# Autodesk Inventor assembly: 한쪽발받침대
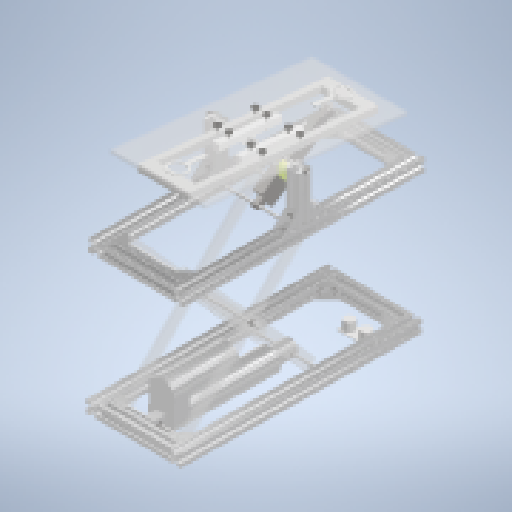
[picture p0: Inventor's stored thumbnail of the model, 512x512]
Saved by Autodesk Inventor 2024 (Build 280153000, 153)
## iProperties
Created: 2024-04-15
Part Number: 한쪽발받침대
Document SubType Name: Assembly
Designer: kkamin5
Mass: 2729.98 g
Surface Area: 7750.02 cm^2
Volume: 1186.1 cm^3
Density: 2.30165 g/cm^3
Author: kkamin5
## Documents named in this file (31)
- C:\Users\kkamin5\OneDrive - UOS\문서\Inventor\EBS project\모델링최종\한쪽발받침대.iam
- C:\Users\kkamin5\OneDrive - UOS\문서\Inventor\EBS project\모델링최종\프로파일_110.ipt
- C:\Users\kkamin5\OneDrive - UOS\문서\Inventor\EBS project\모델링최종\프로파일_380.ipt
- C:\Users\kkamin5\OneDrive - UOS\문서\Inventor\EBS project\모델링최종\t형 슬라이더.ipt
- C:\Users\kkamin5\OneDrive - UOS\문서\Inventor\EBS project\모델링최종\L형 브라켓.ipt
- C:\Users\kkamin5\OneDrive - UOS\문서\Inventor\EBS project\모델링최종\x바.ipt
- C:\Users\kkamin5\OneDrive - UOS\문서\Inventor\EBS project\모델링최종\프로파일_80.ipt
- C:\Users\kkamin5\OneDrive - UOS\문서\Inventor\EBS project\모델링최종\회전체_3d프린트.ipt
- C:\Users\kkamin5\OneDrive - UOS\문서\Inventor\EBS project\모델링최종\발판.ipt
- C:\Users\kkamin5\OneDrive - UOS\문서\Inventor\EBS project\모델링최종\각도엑추에이터브라켓.ipt
- C:\Users\kkamin5\OneDrive - UOS\문서\Inventor\EBS project\모델링최종\120mm 4M 볼트.ipt
- C:\Users\kkamin5\OneDrive - UOS\문서\Inventor\EBS project\모델링최종\볼트M4 10mm.ipt
- C:\Users\kkamin5\OneDrive - UOS\문서\Inventor\EBS project\모델링최종\L브래킷_T슬라이드 볼트조임.iam
- C:\Users\kkamin5\OneDrive - UOS\문서\Inventor\Content Center Files\R2024\ko-KR\BS EN 24035\ISO 4035 - M4BS EN.ipt
- C:\Users\kkamin5\OneDrive - UOS\문서\Inventor\EBS project\모델링최종\M4 볼트 150mm.ipt
- C:\Users\kkamin5\OneDrive - UOS\문서\Inventor\Content Center Files\R2024\ko-KR\ANSI B 18.2.4.1 M(1)\ANSI B 18.2.4.1 M - M4 x 0.7Style 1.ipt
- C:\Users\kkamin5\OneDrive - UOS\문서\Inventor\EBS project\모델링최종\M4 볼트 15mm.ipt
- C:\Users\kkamin5\OneDrive - UOS\문서\Inventor\EBS project\모델링최종\초음파센서.ipt
- C:\Users\kkamin5\OneDrive - UOS\문서\Inventor\EBS project\모델링최종\평기어_가변저항.ipt
- C:\Users\kkamin5\OneDrive - UOS\문서\Inventor\EBS project\모델링최종\각도조절 액추에이터_중간.ipt
- C:\Users\kkamin5\OneDrive - UOS\문서\Inventor\EBS project\모델링최종\높이조절 액추에이터_최소.ipt
- C:\Users\kkamin5\OneDrive - UOS\문서\Inventor\EBS project\모델링최종\압력센서.ipt
- C:\Users\kkamin5\OneDrive - UOS\문서\Inventor\EBS project\모델링최종\가변저항.ipt
- C:\Users\kkamin5\OneDrive - UOS\문서\Inventor\EBS project\모델링최종\초음파센서거리측정용아크릴판.ipt
- C:\Users\kkamin5\OneDrive - UOS\문서\Inventor\EBS project\모델링최종\발판보강지지대2.ipt
- C:\Users\kkamin5\OneDrive - UOS\문서\Inventor\EBS project\모델링최종\한쪽발받침대\AIP\FEA\eo59sf0n4.fins
- C:\Users\kkamin5\OneDrive - UOS\문서\Inventor\EBS project\모델링최종\한쪽발받침대\AIP\FEA\eo59sf0n4.fsat
- C:\Users\kkamin5\OneDrive - UOS\문서\Inventor\EBS project\모델링최종\한쪽발받침대\AIP\FEA\eo59sf0n4.ftes
- C:\Users\kkamin5\OneDrive - UOS\문서\Inventor\EBS project\모델링최종\한쪽발받침대\AIP\FEA\eo59sf0n4.fwiz
- C:\Users\kkamin5\OneDrive - UOS\문서\Inventor\EBS project\모델링최종\한쪽발받침대\AIP\FEA\eo59sf0tc.fmsh
- C:\Users\kkamin5\OneDrive - UOS\문서\Inventor\EBS project\모델링최종\한쪽발받침대\AIP\FEA\eo5b5hja8.fres
## Components (100 placed, 24 different names)
1. 프로파일_110:1 — 메이트:132, 메이트:133, 메이트:134, 메이트:135, 메이트:144
2. 프로파일_380:1 — 메이트:136, 메이트:138, 메이트:148, 플러쉬:34, 플러쉬:52, 메이트:327, 메이트:328
3. 프로파일_110:2 — 메이트:146, 플러쉬:33, 메이트:149, 메이트:265
4. 프로파일_380:2 — 메이트:137, 메이트:147
5. 프로파일_110:3
6. 프로파일_380:3 — 메이트:161, 메이트:162, 메이트:164, 메이트:166, 메이트:190, 메이트:335
7. 프로파일_110:4 — 메이트:189, 플러쉬:40, 메이트:191, 플러쉬:41, 메이트:341
8. 프로파일_380:4 — 메이트:169, 메이트:170, 플러쉬:39, 메이트:176, 메이트:192, 메이트:340
9. t형 슬라이더:1 — 메이트:139
10. t형 슬라이더:2 — 메이트:174
11. t형 슬라이더:3 — 메이트:198
12. t형 슬라이더:4 — 메이트:175
13. t형 슬라이더:5 — 메이트:129
14. t형 슬라이더:6 — 메이트:131
15. x바:1 — 메이트:130, 메이트:160, 메이트:182
16. x바:2 — 메이트:126, 메이트:141, 메이트:159, 메이트:185
17. x바:3 — 메이트:125, 메이트:140, 메이트:188
18. x바:4 — 메이트:128, 메이트:142, 메이트:179
19. t형 슬라이더:7
20. t형 슬라이더:8 — 메이트:163
21. t형 슬라이더:9 — 메이트:173, 플러쉬:42
22. t형 슬라이더:10 — 메이트:172
23. 프로파일_80:1 — 메이트:168, 플러쉬:38, 메이트:171, 플러쉬:42, 플러쉬:47, 메이트:219
24. 프로파일_80:2 — 플러쉬:36, 메이트:165, 메이트:167, 플러쉬:37, 메이트:215, 메이트:217, 메이트:330, 메이트:333, 각도:3, 플러쉬:56
25. L형 브라켓:5 — 메이트:152, 메이트:153, 메이트:154
26. L형 브라켓:6 — 메이트:143, 메이트:156, 메이트:157
27. L형 브라켓:7 — 메이트:237, 메이트:238, 메이트:239
28. L형 브라켓:8 — 메이트:234, 메이트:235, 메이트:236
29. 회전체_3d프린트:1 — 메이트:209, 메이트:311, 메이트:312, 메이트:317, 메이트:318, 메이트:338
30. 발판:1 — 메이트:214, 플러쉬:48, 플러쉬:49, 메이트:269, 메이트:278, 메이트:281, 플러쉬:56, 메이트:344
31. 각도엑추에이터브라켓:1 — 메이트:229, 메이트:245, 메이트:259, 메이트:323
32. 120mm 4M 볼트:1 — 메이트:125, 메이트:126, 메이트:138, 메이트:139, 메이트:184, 메이트:187, 메이트:198, 메이트:256, 메이트:257, 메이트:320
33. 120mm 4M 볼트:2 — 메이트:128, 메이트:129, 메이트:130, 메이트:131, 메이트:136, 메이트:137, 메이트:143, 메이트:178, 메이트:181, 메이트:210, 메이트:211, 메이트:319
34. t형 슬라이더:11 — 메이트:132, 메이트:133, 메이트:158
35. t형 슬라이더:12 — 메이트:134, 메이트:135, 메이트:145
36. 120mm 4M 볼트:3 — 메이트:140, 메이트:141, 메이트:142, 메이트:250, 메이트:251, 메이트:324
37. 볼트M4 10mm:1 — 메이트:144, 메이트:145, 메이트:155, 메이트:157, 메이트:158
38. L브래킷_T슬라이드 볼트조임:1 [sub-assembly] — 메이트:146, 메이트:147, 플러쉬:33
39. L브래킷_T슬라이드 볼트조임:2 [sub-assembly] — 메이트:148, 메이트:149, 플러쉬:34
40. t형 슬라이더:13 — 메이트:152
41. 볼트M4 10mm:2 — 메이트:154
42. BS EN 24035 - 미터 M4:1 — 메이트:153
43. BS EN 24035 - 미터 M4:2 — 메이트:155, 메이트:156
44. 120mm 4M 볼트:4 — 메이트:159, 메이트:162, 메이트:163, 메이트:183, 메이트:186
45. 120mm 4M 볼트:5 — 메이트:160, 메이트:161, 메이트:174, 메이트:175, 메이트:177, 메이트:180
46. L브래킷_T슬라이드 볼트조임:3 [sub-assembly] — 메이트:189, 메이트:190, 플러쉬:40, 메이트:339
47. L브래킷_T슬라이드 볼트조임:4 [sub-assembly] — 메이트:170, 메이트:171, 플러쉬:39
48. L브래킷_T슬라이드 볼트조임:5 [sub-assembly] — 메이트:168, 메이트:169, 플러쉬:38
49. L브래킷_T슬라이드 볼트조임:6 [sub-assembly] — 메이트:166, 메이트:167, 플러쉬:37
50. L브래킷_T슬라이드 볼트조임:7 [sub-assembly] — 메이트:191, 메이트:192, 플러쉬:41
51. L브래킷_T슬라이드 볼트조임:8 [sub-assembly] — 플러쉬:36, 메이트:164, 메이트:165
52. 120mm 4M 볼트:6 — 메이트:172, 메이트:173, 메이트:176, 메이트:321
53. x바:5 — 메이트:177, 메이트:178, 메이트:179, 메이트:252, 메이트:324
54. x바:6 — 메이트:180, 메이트:181, 메이트:182, 메이트:253
55. x바:7 — 메이트:183, 메이트:184, 메이트:185
56. x바:8 — 메이트:186, 메이트:187, 메이트:188
57. M4 볼트 150mm:1 — 메이트:209, 플러쉬:47, 메이트:215, 메이트:216, 메이트:218, 메이트:272
58. 6각 너트 미터 M4 x 0.7:1 — 메이트:211, 메이트:326
59. 6각 너트 미터 M4 x 0.7:2 — 메이트:210, 메이트:325, 메이트:327
60. 발판:2 — 메이트:214, 플러쉬:48, 플러쉬:49, 메이트:284, 메이트:285, 메이트:288, 메이트:289, 메이트:292, 메이트:293, 메이트:296, 메이트:297, 메이트:303, 메이트:304, 메이트:305, 메이트:306, 메이트:307, 메이트:308, 메이트:309, 메이트:310, 메이트:331, 메이트:332, 각도:1, 각도:2
61. 6각 너트 미터 M4 x 0.7:3 — 메이트:218, 메이트:219
62. 6각 너트 미터 M4 x 0.7:4 — 메이트:216, 메이트:217
63. M4 볼트 15mm:5 — 메이트:229, 메이트:244, 메이트:259, 메이트:322
64. t형 슬라이더:14 — 메이트:235
65. 볼트M4 10mm:3 — 메이트:236
66. BS EN 24035 - 미터 M4:3 — 메이트:234
67. t형 슬라이더:15 — 메이트:237
68. 볼트M4 10mm:4 — 메이트:239
69. BS EN 24035 - 미터 M4:4 — 메이트:238
70. BS EN 24035 - 미터 M4:5 — 메이트:244, 메이트:245
71. BS EN 24035 - 미터 M4:10 — 메이트:250, 메이트:253
72. BS EN 24035 - 미터 M4:11 — 메이트:251, 메이트:252
73. BS EN 24035 - 미터 M4:14 — 메이트:256, 메이트:329
74. BS EN 24035 - 미터 M4:15 — 메이트:257, 메이트:328, 메이트:329
75. 초음파센서:2 — 플러쉬:52, 메이트:265
76. 회전체_3d프린트:2 — 메이트:269, 메이트:272, 메이트:278, 메이트:281, 메이트:286, 메이트:290, 메이트:336, 메이트:337
77. M4 볼트 15mm:6 — 메이트:284, 메이트:285
78. BS EN 24035 - 미터 M4:16 — 메이트:286
79. M4 볼트 15mm:7 — 메이트:288, 메이트:289
80. BS EN 24035 - 미터 M4:17 — 메이트:290
81. M4 볼트 15mm:8 — 메이트:292, 메이트:293
82. BS EN 24035 - 미터 M4:18
83. M4 볼트 15mm:9 — 메이트:296, 메이트:297
84. BS EN 24035 - 미터 M4:19
85. M4 볼트 15mm:10 — 메이트:299, 메이트:303, 메이트:307, 메이트:318
86. BS EN 24035 - 미터 M4:20 — 메이트:299, 메이트:311
87. M4 볼트 15mm:11 — 메이트:304, 메이트:308, 메이트:342
88. BS EN 24035 - 미터 M4:21
89. M4 볼트 15mm:12 — 메이트:305, 메이트:309, 메이트:317
90. BS EN 24035 - 미터 M4:22 — 메이트:312
91. M4 볼트 15mm:13 — 메이트:306, 메이트:310, 메이트:343
92. BS EN 24035 - 미터 M4:23
93. 평기어_가변저항:1 — 메이트:330, 메이트:334
94. 각도조절 액추에이터_중간:1 — 메이트:321, 메이트:322, 메이트:323
95. 높이조절 액추에이터_최소:1 — 메이트:319, 메이트:320, 메이트:325, 메이트:326
96. 압력센서:1 — 메이트:332, 각도:2, 플러쉬:55, 메이트:338
97. 압력센서:2 — 메이트:331, 각도:1, 플러쉬:55, 메이트:336, 메이트:337
98. 가변저항:1 — 메이트:333, 메이트:334, 각도:3, 메이트:335
99. 초음파센서거리측정용아크릴판:1 — 메이트:339, 메이트:340, 메이트:341
100. 발판보강지지대2:1 — 메이트:342, 메이트:343, 메이트:344
## Relationships (246: Mate 202, Flush 41, Angle 3)
- [Mate]: 프로파일_110:2 ↔ 프로파일_380:2
- [Flush]: 프로파일_110:2 ↔ 프로파일_380:2
- [Flush]: 프로파일_110:2 ↔ 프로파일_380:2
- [Mate]: 프로파일_380:1 ↔ 프로파일_110:2
- [Flush]: 프로파일_380:1 ↔ 프로파일_110:2
- [Flush]: 프로파일_380:1 ↔ 프로파일_110:2
- [Mate]: 프로파일_110:1 ↔ 프로파일_380:1
- [Flush]: 프로파일_110:1 ↔ 프로파일_380:1
- [Flush]: 프로파일_110:1 ↔ 프로파일_380:1
- [Mate]: 프로파일_110:4 ↔ 프로파일_380:4
- [Flush]: 프로파일_110:4 ↔ 프로파일_380:4
- [Flush]: 프로파일_110:4 ↔ 프로파일_380:4
- [Mate]: 프로파일_380:3 ↔ 프로파일_110:4
- [Flush]: 프로파일_380:3 ↔ 프로파일_110:4
- [Flush]: 프로파일_380:3 ↔ 프로파일_110:4
- [Mate]: 프로파일_110:3 ↔ 프로파일_380:3
- [Flush]: 프로파일_110:3 ↔ 프로파일_380:3
- [Flush]: 프로파일_110:3 ↔ 프로파일_380:3
- [Mate] (0.4 mm): 프로파일_380:4 ↔ t형 슬라이더:4
- [Mate] (0.1 mm): 프로파일_380:4 ↔ t형 슬라이더:4
- [Mate] (0.4 mm): 프로파일_380:2 ↔ t형 슬라이더:3
- [Mate] (0.2 mm): 프로파일_380:2 ↔ t형 슬라이더:3
- [Mate] (0.4 mm): 프로파일_380:3 ↔ t형 슬라이더:2
- [Mate] (0.1 mm): 프로파일_380:3 ↔ t형 슬라이더:2
- [Mate] (0.4 mm): 프로파일_380:1 ↔ t형 슬라이더:1
- [Mate]: 프로파일_380:1 ↔ t형 슬라이더:1
- [Flush]: 프로파일_110:1 ↔ 프로파일_110:3
- [Flush]: 프로파일_380:1 ↔ 프로파일_380:3
- [Mate] (0.4 mm): 프로파일_380:2 ↔ t형 슬라이더:6
- [Mate] (0.1 mm): 프로파일_380:2 ↔ t형 슬라이더:6
- [Mate] (0.4 mm): 프로파일_380:1 ↔ t형 슬라이더:5
- [Mate] (0.1 mm): 프로파일_380:1 ↔ t형 슬라이더:5
- [Mate]: x바:1 ↔ x바:4
- [Mate] (10 mm): 프로파일_380:4 ↔ x바:1
- [Mate] (10 mm): 프로파일_380:3 ↔ x바:4
- [Mate] (0.4 mm): 프로파일_380:4 ↔ t형 슬라이더:7
- [Mate]: 프로파일_380:4 ↔ t형 슬라이더:7
- [Mate]: 프로파일_380:3 ↔ t형 슬라이더:8
- [Mate]: 프로파일_380:3 ↔ t형 슬라이더:8
- [Flush]: t형 슬라이더:6 ↔ t형 슬라이더:7
- [Mate] (14 mm): 프로파일_380:1 ↔ x바:3
- [Mate] (14 mm): 프로파일_380:2 ↔ x바:2
- [Mate]: 프로파일_380:4 ↔ t형 슬라이더:9
- [Mate] (0.4 mm): 프로파일_380:4 ↔ t형 슬라이더:9
- [Mate]: 프로파일_380:3 ↔ t형 슬라이더:10
- [Mate] (0.4 mm): 프로파일_380:3 ↔ t형 슬라이더:10
- [Mate]: 프로파일_380:3 ↔ 프로파일_80:2
- [Mate]: 프로파일_380:4 ↔ 프로파일_80:1
- [Flush]: 프로파일_380:4 ↔ 프로파일_80:1
- [Flush]: 프로파일_380:3 ↔ 프로파일_80:2
- [Flush] (180 mm): 프로파일_380:4 ↔ 프로파일_80:1
- [Flush] (5 mm): t형 슬라이더:10 ↔ 프로파일_80:2
- [Mate]: 프로파일_380:2 ↔ L형 브라켓:5
- [Flush] (1.5 mm): 프로파일_110:1 ↔ L형 브라켓:5
- [Mate]: 프로파일_110:1 ↔ L형 브라켓:5
- [Mate]: 프로파일_380:1 ↔ L형 브라켓:6
- [Flush] (1.5 mm): 프로파일_110:1 ↔ L형 브라켓:6
- [Mate]: 프로파일_110:1 ↔ L형 브라켓:6
- [Flush] (1.5 mm): 프로파일_110:3 ↔ L형 브라켓:7
- [Mate]: 프로파일_380:3 ↔ L형 브라켓:7
- [Mate]: 프로파일_110:3 ↔ L형 브라켓:7
- [Flush] (1.5 mm): 프로파일_110:3 ↔ L형 브라켓:8
- [Mate]: 프로파일_110:3 ↔ L형 브라켓:8
- [Mate]: 프로파일_380:4 ↔ L형 브라켓:8
- [Mate]: 회전체_3d프린트:1 ↔ 발판:1
- [Mate]: 발판:1 ↔ 각도엑추에이터브라켓:1
- [Mate]: 발판:1 ↔ 각도엑추에이터브라켓:1
- 메이트:125 [Mate]: x바:3 ↔ 120mm 4M 볼트:1
- 메이트:126 [Mate]: x바:2 ↔ 120mm 4M 볼트:1
- 메이트:128 [Mate]: x바:4 ↔ 120mm 4M 볼트:2
- 메이트:129 [Mate]: t형 슬라이더:5 ↔ 120mm 4M 볼트:2
- 메이트:130 [Mate]: x바:1 ↔ 120mm 4M 볼트:2
- 메이트:131 [Mate]: t형 슬라이더:6 ↔ 120mm 4M 볼트:2
- 메이트:132 [Mate] (0.1 mm): 프로파일_110:1 ↔ t형 슬라이더:11
- 메이트:133 [Mate] (0.4 mm): 프로파일_110:1 ↔ t형 슬라이더:11
- 메이트:134 [Mate] (0.4 mm): 프로파일_110:1 ↔ t형 슬라이더:12
- 메이트:135 [Mate] (0.1 mm): 프로파일_110:1 ↔ t형 슬라이더:12
- 메이트:136 [Mate] (1 mm): 프로파일_380:1 ↔ 120mm 4M 볼트:2
- 메이트:137 [Mate] (1 mm): 프로파일_380:2 ↔ 120mm 4M 볼트:2
- 메이트:138 [Mate] (1 mm): 프로파일_380:1 ↔ 120mm 4M 볼트:1
- 메이트:139 [Mate]: t형 슬라이더:1 ↔ 120mm 4M 볼트:1
- 메이트:140 [Mate]: x바:3 ↔ 120mm 4M 볼트:3
- 메이트:141 [Mate]: x바:2 ↔ 120mm 4M 볼트:3
- 메이트:142 [Mate]: x바:4 ↔ 120mm 4M 볼트:3
- 메이트:143 [Mate]: L형 브라켓:6 ↔ 120mm 4M 볼트:2
- 메이트:144 [Mate]: 프로파일_110:1 ↔ 볼트M4 10mm:1
- 메이트:145 [Mate]: t형 슬라이더:12 ↔ 볼트M4 10mm:1
- 메이트:146 [Mate]: 프로파일_110:2 ↔ L브래킷_T슬라이드 볼트조임:1
- 메이트:147 [Mate]: 프로파일_380:2 ↔ L브래킷_T슬라이드 볼트조임:1
- 플러쉬:33 [Flush] (1.5 mm): 프로파일_110:2 ↔ L브래킷_T슬라이드 볼트조임:1
- 메이트:148 [Mate]: 프로파일_380:1 ↔ L브래킷_T슬라이드 볼트조임:2
- 메이트:149 [Mate]: 프로파일_110:2 ↔ L브래킷_T슬라이드 볼트조임:2
- 플러쉬:34 [Flush] (1.5 mm): 프로파일_380:1 ↔ L브래킷_T슬라이드 볼트조임:2
- [Mate]: t형 슬라이더:13 ↔ 볼트M4 10mm:2
- [Flush]: t형 슬라이더:13 ↔ 볼트M4 10mm:2
- [Mate]: 볼트M4 10mm:2 ↔ BS EN 24035 - 미터 M4:1
- 메이트:152 [Mate] (1.6 mm): L형 브라켓:5 ↔ t형 슬라이더:13
- 메이트:153 [Mate]: L형 브라켓:5 ↔ BS EN 24035 - 미터 M4:1
- 메이트:154 [Mate]: L형 브라켓:5 ↔ 볼트M4 10mm:2
- 메이트:155 [Mate]: 볼트M4 10mm:1 ↔ BS EN 24035 - 미터 M4:2
- 메이트:156 [Mate]: L형 브라켓:6 ↔ BS EN 24035 - 미터 M4:2
- 메이트:157 [Mate]: L형 브라켓:6 ↔ 볼트M4 10mm:1
- 메이트:158 [Mate]: t형 슬라이더:11 ↔ 볼트M4 10mm:1
- 메이트:159 [Mate]: x바:2 ↔ 120mm 4M 볼트:4
- 메이트:160 [Mate]: x바:1 ↔ 120mm 4M 볼트:5
- 메이트:161 [Mate] (1 mm): 프로파일_380:3 ↔ 120mm 4M 볼트:5
- 메이트:162 [Mate] (1 mm): 프로파일_380:3 ↔ 120mm 4M 볼트:4
- 메이트:163 [Mate]: t형 슬라이더:8 ↔ 120mm 4M 볼트:4
- 플러쉬:36 [Flush] (1.5 mm): 프로파일_80:2 ↔ L브래킷_T슬라이드 볼트조임:8
- 메이트:164 [Mate]: 프로파일_380:3 ↔ L브래킷_T슬라이드 볼트조임:8
- 메이트:165 [Mate]: 프로파일_80:2 ↔ L브래킷_T슬라이드 볼트조임:8
- 메이트:166 [Mate]: 프로파일_380:3 ↔ L브래킷_T슬라이드 볼트조임:6
- 메이트:167 [Mate]: 프로파일_80:2 ↔ L브래킷_T슬라이드 볼트조임:6
- 플러쉬:37 [Flush] (1.5 mm): 프로파일_80:2 ↔ L브래킷_T슬라이드 볼트조임:6
- 메이트:168 [Mate]: 프로파일_80:1 ↔ L브래킷_T슬라이드 볼트조임:5
- 메이트:169 [Mate]: 프로파일_380:4 ↔ L브래킷_T슬라이드 볼트조임:5
- 플러쉬:38 [Flush] (1.5 mm): 프로파일_80:1 ↔ L브래킷_T슬라이드 볼트조임:5
- 메이트:170 [Mate]: 프로파일_380:4 ↔ L브래킷_T슬라이드 볼트조임:4
- 메이트:171 [Mate]: 프로파일_80:1 ↔ L브래킷_T슬라이드 볼트조임:4
- 플러쉬:39 [Flush] (1.5 mm): 프로파일_380:4 ↔ L브래킷_T슬라이드 볼트조임:4
- 메이트:172 [Mate]: t형 슬라이더:10 ↔ 120mm 4M 볼트:6
- 메이트:173 [Mate]: t형 슬라이더:9 ↔ 120mm 4M 볼트:6
- 메이트:174 [Mate]: t형 슬라이더:2 ↔ 120mm 4M 볼트:5
- 메이트:175 [Mate]: t형 슬라이더:4 ↔ 120mm 4M 볼트:5
- 메이트:176 [Mate] (1 mm): 프로파일_380:4 ↔ 120mm 4M 볼트:6
- 메이트:177 [Mate]: 120mm 4M 볼트:5 ↔ x바:5
- 메이트:178 [Mate]: 120mm 4M 볼트:2 ↔ x바:5
- 메이트:179 [Mate]: x바:4 ↔ x바:5
- 메이트:180 [Mate]: 120mm 4M 볼트:5 ↔ x바:6
- 메이트:181 [Mate]: 120mm 4M 볼트:2 ↔ x바:6
- 메이트:182 [Mate]: x바:1 ↔ x바:6
- 메이트:183 [Mate]: 120mm 4M 볼트:4 ↔ x바:7
- 메이트:184 [Mate]: 120mm 4M 볼트:1 ↔ x바:7
- 메이트:185 [Mate]: x바:2 ↔ x바:7
- 메이트:186 [Mate]: 120mm 4M 볼트:4 ↔ x바:8
- 메이트:187 [Mate]: 120mm 4M 볼트:1 ↔ x바:8
- 메이트:188 [Mate]: x바:3 ↔ x바:8
- 메이트:189 [Mate]: 프로파일_110:4 ↔ L브래킷_T슬라이드 볼트조임:3
- 메이트:190 [Mate]: 프로파일_380:3 ↔ L브래킷_T슬라이드 볼트조임:3
- 플러쉬:40 [Flush] (1.5 mm): 프로파일_110:4 ↔ L브래킷_T슬라이드 볼트조임:3
- 메이트:191 [Mate]: 프로파일_110:4 ↔ L브래킷_T슬라이드 볼트조임:7
- 메이트:192 [Mate]: 프로파일_380:4 ↔ L브래킷_T슬라이드 볼트조임:7
- 플러쉬:41 [Flush] (1.5 mm): 프로파일_110:4 ↔ L브래킷_T슬라이드 볼트조임:7
- 플러쉬:42 [Flush] (5 mm): t형 슬라이더:9 ↔ 프로파일_80:1
- 메이트:198 [Mate]: t형 슬라이더:3 ↔ 120mm 4M 볼트:1
- 메이트:209 [Mate]: 회전체_3d프린트:1 ↔ M4 볼트 150mm:1
- 플러쉬:47 [Flush] (-5 mm): 프로파일_80:1 ↔ M4 볼트 150mm:1
- 메이트:210 [Mate]: 120mm 4M 볼트:2 ↔ 6각 너트 미터 M4 x 0.7:2
- 메이트:211 [Mate]: 120mm 4M 볼트:2 ↔ 6각 너트 미터 M4 x 0.7:1
- 메이트:214 [Mate]: 발판:1 ↔ 발판:2
- 플러쉬:48 [Flush]: 발판:1 ↔ 발판:2
- 플러쉬:49 [Flush]: 발판:1 ↔ 발판:2
- 메이트:215 [Mate]: 프로파일_80:2 ↔ M4 볼트 150mm:1
- 메이트:216 [Mate]: M4 볼트 150mm:1 ↔ 6각 너트 미터 M4 x 0.7:4
- 메이트:217 [Mate]: 프로파일_80:2 ↔ 6각 너트 미터 M4 x 0.7:4
- 메이트:218 [Mate]: M4 볼트 150mm:1 ↔ 6각 너트 미터 M4 x 0.7:3
- 메이트:219 [Mate]: 프로파일_80:1 ↔ 6각 너트 미터 M4 x 0.7:3
- 메이트:229 [Mate]: 각도엑추에이터브라켓:1 ↔ M4 볼트 15mm:5
- [Mate]: t형 슬라이더:14 ↔ 볼트M4 10mm:3
- [Flush]: t형 슬라이더:14 ↔ 볼트M4 10mm:3
- [Mate]: 볼트M4 10mm:3 ↔ BS EN 24035 - 미터 M4:3
- [Mate]: t형 슬라이더:15 ↔ 볼트M4 10mm:4
- [Flush]: t형 슬라이더:15 ↔ 볼트M4 10mm:4
- [Mate]: 볼트M4 10mm:4 ↔ BS EN 24035 - 미터 M4:4
- 메이트:234 [Mate]: L형 브라켓:8 ↔ BS EN 24035 - 미터 M4:3
- 메이트:235 [Mate] (1.6 mm): L형 브라켓:8 ↔ t형 슬라이더:14
- 메이트:236 [Mate]: L형 브라켓:8 ↔ 볼트M4 10mm:3
- 메이트:237 [Mate] (1.6 mm): L형 브라켓:7 ↔ t형 슬라이더:15
- 메이트:238 [Mate]: L형 브라켓:7 ↔ BS EN 24035 - 미터 M4:4
- 메이트:239 [Mate]: L형 브라켓:7 ↔ 볼트M4 10mm:4
- 메이트:244 [Mate]: M4 볼트 15mm:5 ↔ BS EN 24035 - 미터 M4:5
- 메이트:245 [Mate]: 각도엑추에이터브라켓:1 ↔ BS EN 24035 - 미터 M4:5
- 메이트:250 [Mate]: 120mm 4M 볼트:3 ↔ BS EN 24035 - 미터 M4:10
- 메이트:251 [Mate]: 120mm 4M 볼트:3 ↔ BS EN 24035 - 미터 M4:11
- 메이트:252 [Mate]: x바:5 ↔ BS EN 24035 - 미터 M4:11
- 메이트:253 [Mate]: x바:6 ↔ BS EN 24035 - 미터 M4:10
- 메이트:256 [Mate]: 120mm 4M 볼트:1 ↔ BS EN 24035 - 미터 M4:14
- 메이트:257 [Mate]: 120mm 4M 볼트:1 ↔ BS EN 24035 - 미터 M4:15
- 메이트:259 [Mate]: 각도엑추에이터브라켓:1 ↔ M4 볼트 15mm:5
- 플러쉬:52 [Flush] (-23 mm): 프로파일_380:1 ↔ 초음파센서:2
- 메이트:265 [Mate]: 프로파일_110:2 ↔ 초음파센서:2
- 메이트:269 [Mate]: 발판:1 ↔ 회전체_3d프린트:2
- 메이트:272 [Mate]: M4 볼트 150mm:1 ↔ 회전체_3d프린트:2
- 메이트:278 [Mate]: 발판:1 ↔ 회전체_3d프린트:2
- 메이트:281 [Mate]: 발판:1 ↔ 회전체_3d프린트:2
- [Mate]: M4 볼트 15mm:6 ↔ BS EN 24035 - 미터 M4:16
- 메이트:284 [Mate]: 발판:2 ↔ M4 볼트 15mm:6
- 메이트:285 [Mate]: 발판:2 ↔ M4 볼트 15mm:6
- 메이트:286 [Mate]: 회전체_3d프린트:2 ↔ BS EN 24035 - 미터 M4:16
- [Mate]: M4 볼트 15mm:7 ↔ BS EN 24035 - 미터 M4:17
- 메이트:288 [Mate]: 발판:2 ↔ M4 볼트 15mm:7
- 메이트:289 [Mate]: 발판:2 ↔ M4 볼트 15mm:7
- 메이트:290 [Mate]: 회전체_3d프린트:2 ↔ BS EN 24035 - 미터 M4:17
- [Mate]: M4 볼트 15mm:8 ↔ BS EN 24035 - 미터 M4:18
- 메이트:292 [Mate]: 발판:2 ↔ M4 볼트 15mm:8
- 메이트:293 [Mate]: 발판:2 ↔ M4 볼트 15mm:8
- [Mate]: M4 볼트 15mm:9 ↔ BS EN 24035 - 미터 M4:19
- 메이트:296 [Mate]: 발판:2 ↔ M4 볼트 15mm:9
- 메이트:297 [Mate]: 발판:2 ↔ M4 볼트 15mm:9
- 메이트:299 [Mate]: M4 볼트 15mm:10 ↔ BS EN 24035 - 미터 M4:20
- [Mate]: M4 볼트 15mm:11 ↔ BS EN 24035 - 미터 M4:21
- [Mate]: M4 볼트 15mm:12 ↔ BS EN 24035 - 미터 M4:22
- [Mate]: M4 볼트 15mm:13 ↔ BS EN 24035 - 미터 M4:23
- 메이트:303 [Mate]: 발판:2 ↔ M4 볼트 15mm:10
- 메이트:304 [Mate]: 발판:2 ↔ M4 볼트 15mm:11
- 메이트:305 [Mate]: 발판:2 ↔ M4 볼트 15mm:12
- 메이트:306 [Mate]: 발판:2 ↔ M4 볼트 15mm:13
- 메이트:307 [Mate]: 발판:2 ↔ M4 볼트 15mm:10
- 메이트:308 [Mate]: 발판:2 ↔ M4 볼트 15mm:11
- 메이트:309 [Mate]: 발판:2 ↔ M4 볼트 15mm:12
- 메이트:310 [Mate]: 발판:2 ↔ M4 볼트 15mm:13
- 메이트:311 [Mate]: 회전체_3d프린트:1 ↔ BS EN 24035 - 미터 M4:20
- 메이트:312 [Mate]: 회전체_3d프린트:1 ↔ BS EN 24035 - 미터 M4:22
- 메이트:317 [Mate]: 회전체_3d프린트:1 ↔ M4 볼트 15mm:12
- 메이트:318 [Mate]: 회전체_3d프린트:1 ↔ M4 볼트 15mm:10
- 메이트:319 [Mate]: 120mm 4M 볼트:2 ↔ 높이조절 액추에이터_최소:1
- 메이트:320 [Mate]: 120mm 4M 볼트:1 ↔ 높이조절 액추에이터_최소:1
- 메이트:321 [Mate]: 120mm 4M 볼트:6 ↔ 각도조절 액추에이터_중간:1
- 메이트:322 [Mate]: M4 볼트 15mm:5 ↔ 각도조절 액추에이터_중간:1
- 메이트:323 [Mate]: 각도엑추에이터브라켓:1 ↔ 각도조절 액추에이터_중간:1
- 메이트:324 [Mate]: 120mm 4M 볼트:3 ↔ x바:5
- 메이트:325 [Mate]: 6각 너트 미터 M4 x 0.7:2 ↔ 높이조절 액추에이터_최소:1
- 메이트:326 [Mate]: 6각 너트 미터 M4 x 0.7:1 ↔ 높이조절 액추에이터_최소:1
- 메이트:327 [Mate] (44.3 mm): 프로파일_380:1 ↔ 6각 너트 미터 M4 x 0.7:2
- 메이트:328 [Mate] (40.3 mm): 프로파일_380:1 ↔ BS EN 24035 - 미터 M4:15
- 메이트:329 [Mate] (25 mm): BS EN 24035 - 미터 M4:14 ↔ BS EN 24035 - 미터 M4:15
- 메이트:330 [Mate] (-10 mm): 프로파일_80:2 ↔ 평기어_가변저항:1
- 메이트:331 [Mate]: 발판:2 ↔ 압력센서:2
- 메이트:332 [Mate]: 발판:2 ↔ 압력센서:1
- 각도:1 [Angle] (0 deg): 발판:2 ↔ 압력센서:2
- 각도:2 [Angle] (0 deg): 발판:2 ↔ 압력센서:1
- 플러쉬:55 [Flush]: 압력센서:1 ↔ 압력센서:2
- 메이트:333 [Mate]: 프로파일_80:2 ↔ 가변저항:1
- 메이트:334 [Mate]: 평기어_가변저항:1 ↔ 가변저항:1
- 각도:3 [Angle] (0 deg): 프로파일_80:2 ↔ 가변저항:1
- 플러쉬:56 [Flush]: 프로파일_80:2 ↔ 발판:1
- 메이트:335 [Mate] (54.1 mm): 프로파일_380:3 ↔ 가변저항:1
- 메이트:336 [Mate] (35 mm): 회전체_3d프린트:2 ↔ 압력센서:2
- 메이트:337 [Mate] (10 mm): 회전체_3d프린트:2 ↔ 압력센서:2
- 메이트:338 [Mate] (35 mm): 회전체_3d프린트:1 ↔ 압력센서:1
- 메이트:339 [Mate]: L브래킷_T슬라이드 볼트조임:3 ↔ 초음파센서거리측정용아크릴판:1
- 메이트:340 [Mate]: 프로파일_380:4 ↔ 초음파센서거리측정용아크릴판:1
- 메이트:341 [Mate]: 프로파일_110:4 ↔ 초음파센서거리측정용아크릴판:1
- 메이트:342 [Mate]: M4 볼트 15mm:11 ↔ 발판보강지지대2:1
- 메이트:343 [Mate]: M4 볼트 15mm:13 ↔ 발판보강지지대2:1
- 메이트:344 [Mate]: 발판:1 ↔ 발판보강지지대2:1
## Named parameters: d440_d68 = 0 mm, d441_d69 = 10 mm, d442_d70 = 10 mm, d444_d72 = 0.4 mm, d445_d73 = 0 mm, d447_d75 = 0 mm, d448_d76 = 0 mm, d451_d8 = 0 mm, d452_d9 = 0 mm, d453_d10 = 0 mm, d454_d11_d2 = 0 mm, d455_d12_d3 = 0 mm, d456_d13_d4 = 0 mm, d457_d14_d5 = 0 mm, d458_d15_d6 = 0 mm, d459_d16_d7 = 0 mm, d460_d17_d8 = 0 mm, d461_d18_d9 = 0 mm, d462_d19_d10 = 0 mm, d463_d33 = 0.4 mm, d464_d34 = 0.1 mm, d465_d35 = 0.4 mm, d466_d36 = 0.2 mm, d467_d37 = 0.4 mm, d468_d38 = 0.1 mm, d469_d39 = 0.4 mm, d470_d40 = 0 mm, d475_d2 = 0 mm, d476_d3 = 0 mm, d477_d4 = 0 mm, d478_d5 = 0 mm, d479_d6 = 0 mm, d480_d7 = 0 mm, d499_d182 = 0 mm, d500_d183 = 1.5 mm, d501_d184 = 0 mm, d502_d185 = 0 mm, d503_d186 = 1.5 mm, d504_d187 = 0 mm, d506_d189 = 1.5 mm, d507_d190 = 0 mm, d508_d191 = 0 mm, d509_d192 = 1.5 mm, d510_d193 = 0 mm, d511_d194 = 0 mm, d514_d197 = 0 mm, d522_d129 = 0 mm, d523_d130 = 0.4 mm, d530_d137 = 0 mm, d531_d138 = 0.4 mm, d532_d385 = 0 mm, d535_d151 = 0 mm, d536_d152 = 0 mm, d537_d153 = 0 mm, d538_d154 = 0 mm, d556_d205 = 0 mm, d391_d178 = 180 mm, d392_d179 = 5 mm, d403_d80 = 0 mm, d408_d85 = 14 mm, d409_d86 = 14 mm, d421_d47 = 0 mm, d422_d48 = 0 mm, d423_d49 = 0.4 mm, d424_d50 = 0.1 mm, d425_d51 = 0.4 mm, d426_d52 = 0.1 mm, sa_0 = 15000, d303_d1 = 0 mm, d304_d7 = 0 mm, d305_d10 = 0 mm, d306_d1 = 0 mm, d307_d7 = 0 mm, d308_d10 = 0 mm, d377_d317 = 0 mm, d381_d317 = 0 mm, d385_d317 = 0 mm, d389_d317 = 0 mm, d394_d393 = 0 mm, d395_d393 = 0 mm, d396_d393 = 0 mm
note: some values were not read from the file. Shown as the stored number, unit unknown: "sa_0".
